# Autodesk Inventor assembly: 200-02-ROCKER-CONNECTOR-ASM-R
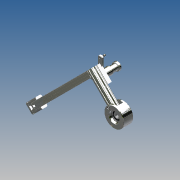
[picture p0: Inventor's stored thumbnail of the model, 180x180]
Saved by Autodesk Inventor 2018.2 (Build 222227000, 227)
## iProperties
Manager: feesmrt
Company: FRANCOR
Created: 2017-12-19
Part Number: 200-02-ROCKER-CONNECTOR-ASM-R
Project: Rescue Robot
Cost Center: -
Material: Generisch
Document SubType Name: Assembly
Designer: feesmrt
Engineer: feesmrt
Authority: feesmrt
Description: Rocker Connector Right Side ASM
Stock Number: 200-02-ROCKER-CONNECTOR-ASM-R
Subject: Rescue Robot
Author: feesmrt
Revision Number: 1
Title: Rocker Connector Right Side ASM
## Documents named in this file (6)
- D:\Programmierung\FRANC0R\CAD\02-Rocker-Bogie-Robot\200-ROCKER-BOGIE\200-02-ROCKER-CONNECTOR-ASM-R.iam
- D:\Programmierung\FRANC0R\CAD\02-Rocker-Bogie-Robot\200-ROCKER-BOGIE\200-20-ROCKER-CONNECTOR\200-20-ROCKER-CONNECTOR-ASM-01.iam
- D:\Programmierung\FRANC0R\CAD\02-Rocker-Bogie-Robot\200-ROCKER-BOGIE\200-30-BOGIE-BEARING\200-30-BOGIE-BEARING-ASM-01.iam
- D:\Programmierung\FRANC0R\CAD\02-Rocker-Bogie-Robot\200-ROCKER-BOGIE\200-50-WHEEL-CONNECTOR\200-50-WHEEL-CONNECTOR-30MM-ASM-01.iam
- D:\Programmierung\FRANC0R\CAD\02-Rocker-Bogie-Robot\200-ROCKER-BOGIE\200-20-ROCKER-CONNECTOR\200-20-ROCKER-CONNECTOR-P-01.ipt
- D:\Programmierung\FRANC0R\CAD\02-Rocker-Bogie-Robot\200-ROCKER-BOGIE\200-20-ROCKER-CONNECTOR\200-20-ROCKER-CONNECTOR-P-02.ipt
## Components (5 placed, 5 different names)
1. 200-20-ROCKER-CONNECTOR-ASM-01:1 [sub-assembly] — Passend:2, Fluchtend:1, Fluchtend:2, Passend:4, Fluchtend:3
2. 200-30-BOGIE-BEARING-ASM-01:1 [sub-assembly] — Passend:1, Passend:5, Fluchtend:4
3. 200-50-WHEEL-CONNECTOR-30MM-ASM-01:1 [sub-assembly] — Passend:6, Passend:7, Fluchtend:5
4. 200-20-ROCKER-CONNECTOR-P-01:1 — Passend:1, Passend:2, Fluchtend:1, Fluchtend:2, Passend:3, Passend:5, Fluchtend:4
5. 200-20-ROCKER-CONNECTOR-P-02:1 — Passend:3, Passend:4, Fluchtend:3, Passend:6, Passend:7, Fluchtend:5
## Relationships (12: Mate 7, Flush 5)
- Passend:1 [Mate]: 200-30-BOGIE-BEARING-ASM-01:1 ↔ 200-20-ROCKER-CONNECTOR-P-01:1
- Passend:2 [Mate]: 200-20-ROCKER-CONNECTOR-ASM-01:1 ↔ 200-20-ROCKER-CONNECTOR-P-01:1
- Fluchtend:1 [Flush]: 200-20-ROCKER-CONNECTOR-ASM-01:1 ↔ 200-20-ROCKER-CONNECTOR-P-01:1
- Fluchtend:2 [Flush]: 200-20-ROCKER-CONNECTOR-ASM-01:1 ↔ 200-20-ROCKER-CONNECTOR-P-01:1
- Passend:3 [Mate]: 200-20-ROCKER-CONNECTOR-P-01:1 ↔ 200-20-ROCKER-CONNECTOR-P-02:1
- Passend:4 [Mate]: 200-20-ROCKER-CONNECTOR-ASM-01:1 ↔ 200-20-ROCKER-CONNECTOR-P-02:1
- Fluchtend:3 [Flush]: 200-20-ROCKER-CONNECTOR-ASM-01:1 ↔ 200-20-ROCKER-CONNECTOR-P-02:1
- Passend:5 [Mate]: 200-30-BOGIE-BEARING-ASM-01:1 ↔ 200-20-ROCKER-CONNECTOR-P-01:1
- Fluchtend:4 [Flush]: 200-30-BOGIE-BEARING-ASM-01:1 ↔ 200-20-ROCKER-CONNECTOR-P-01:1
- Passend:6 [Mate]: 200-50-WHEEL-CONNECTOR-30MM-ASM-01:1 ↔ 200-20-ROCKER-CONNECTOR-P-02:1
- Passend:7 [Mate]: 200-50-WHEEL-CONNECTOR-30MM-ASM-01:1 ↔ 200-20-ROCKER-CONNECTOR-P-02:1
- Fluchtend:5 [Flush]: 200-50-WHEEL-CONNECTOR-30MM-ASM-01:1 ↔ 200-20-ROCKER-CONNECTOR-P-02:1
